# Autodesk Inventor assembly: Assembly
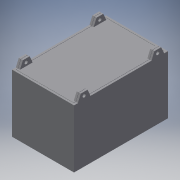
[picture p0: Inventor's stored thumbnail of the model, 180x180]
Saved by Autodesk Inventor 2016 (Build 200138000, 138)
## iProperties
Created: 2018-01-17
Part Number: Assembly
Document SubType Name: Assembly
Designer: trevo
Author: trevo
## Documents named in this file (3)
- D:\GitHub\CoffeeTrackerPro\Logging Device\Housing for Filter\Assembly.iam
- D:\GitHub\CoffeeTrackerPro\Logging Device\Housing for Filter\Housing for Filter.ipt
- D:\GitHub\CoffeeTrackerPro\Logging Device\Housing for Filter\Pi Holder.ipt
## Components (2 placed, 2 different names)
1. Housing for Filter:1 — Mate:1, Mate:2, Flush:1
2. Pi Holder:1 — Mate:1, Mate:2, Flush:1
## Relationships (3: Mate 2, Flush 1)
- Mate:1 (0.25 mm): Housing for Filter:1 ↔ Pi Holder:1
- Mate:2 (0.25 mm): Housing for Filter:1 ↔ Pi Holder:1
- Flush:1: Housing for Filter:1 ↔ Pi Holder:1
